# Autodesk Inventor assembly: front
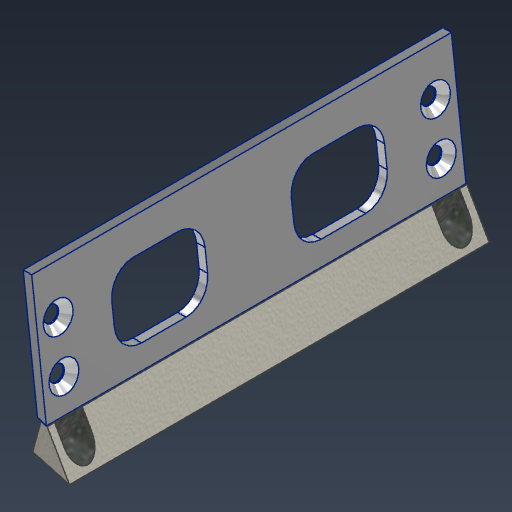
[picture p0: Inventor's stored thumbnail of the model, 512x512]
Saved by Autodesk Inventor 2023 (Build 270158000, 158)
## iProperties
Created: 2025-04-06
Part Number: front
Document SubType Name: Assembly
Designer: szymo
Author: szymo
## Documents named in this file (3)
- D:\tech\robotyka\robots\evangelion\inventor-project\front.iam
- D:\tech\robotyka\robots\evangelion\inventor-project\plog.ipt
- D:\tech\robotyka\robots\evangelion\inventor-project\front-plate.ipt
## Components (2 placed, 2 different names)
1. plog:1 — Flush:1
2. front-plate:1 — Flush:1
## Relationships (1: Flush 1)
- Flush:1: plog:1 ↔ front-plate:1
